# Autodesk Inventor assembly: Sistema movimiento derecho
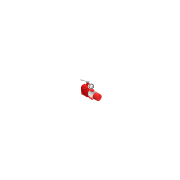
[picture p0: Inventor's stored thumbnail of the model, 180x180]
Saved by Autodesk Inventor 2021 (Build 250183000, 183)
## iProperties
Created: 2021-06-19
Part Number: Sistema movimiento derecho
Document SubType Name: Assembly
Designer: Andrés Holguín
Author: Andrés Holguín
## Documents named in this file (9)
- C:\Users\Santiago Suárez\Documents\GitHub\Dis.-Mecatronico-E6\inventor proyecto\Motores y reductores\Sistema movimiento derecho.iam
- C:\Users\Santiago Suárez\Documents\GitHub\Dis.-Mecatronico-E6\inventor proyecto\Motores y reductores\Reductor Derecha.iam
- Reductor Derecha.iam
- C:\Users\Santiago Suárez\Documents\GitHub\Dis.-Mecatronico-E6\inventor proyecto\Motores y reductores\pasador.ipt
- C:\Users\Santiago Suárez\Documents\GitHub\Dis.-Mecatronico-E6\inventor proyecto\Motores y reductores\Biela Completa.iam
- C:\Users\Santiago Suárez\Documents\GitHub\Dis.-Mecatronico-E6\inventor proyecto\Motores y reductores\placa manivela.ipt
- C:\Users\Santiago Suárez\Documents\Inventor\Content Center Files\R2021\en-US\AS 1421(4)\AS 1421 - M16 x 16 Flat Point.ipt
- C:\Users\Santiago Suárez\Documents\Inventor\Content Center Files\R2021\en-US\AS 2465(3)\AS 2465 - 1  UNC(2).ipt
- C:\Users\Santiago Suárez\Documents\GitHub\Dis.-Mecatronico-E6\inventor proyecto\Motores y reductores\Frame\132s_5.iam
## Components (7 placed, 7 different names)
1. Reductor Derecha:1 [sub-assembly] — 25, Mate:1, Rigid:4
2. pasador:1 — Insert:2, Insert:3, Rotational:1
3. Biela Completa:1 [sub-assembly] — Insert:3
4. placa manivela:1 — 25, Mate:1, Insert:2, Rigid:5
5. 132s_5:1 [sub-assembly] — Rigid:4
6. AS 1421 Flat Point - Metric M16 x 16 Flat Point:2 — Rigid:5
7. AS 2465 (Unified hexagon bolts, screws and nuts (UNC and UNF threads) - Inch 1  UNC:2 — Rotational:1
## Relationships (7: Insert 3, WeldJoint 2, Mate 1, RevoluteJoint 1)
- 25 [Insert] (35 mm): Reductor Derecha:1 ↔ placa manivela:1
- Mate:1: Reductor Derecha:1 ↔ placa manivela:1
- Insert:2: pasador:1 ↔ placa manivela:1
- Insert:3 (20 mm): pasador:1 ↔ Biela Completa:1
- Rigid:4 [WeldJoint]: Reductor Derecha:1 ↔ 132s_5:1
- Rotational:1 [RevoluteJoint]: pasador:1 ↔ AS 2465 (Unified hexagon bolts, screws and nuts (UNC and UNF threads) - Inch 1  UNC:2
- Rigid:5 [WeldJoint]: placa manivela:1 ↔ AS 1421 Flat Point - Metric M16 x 16 Flat Point:2
